# Autodesk Inventor assembly: estação_bga
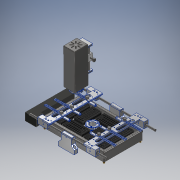
[picture p0: Inventor's stored thumbnail of the model, 180x180]
Saved by Autodesk Inventor 2018 (Build 220112000, 112)
## iProperties
Created: 2018-05-03
Part Number: estação_bga
Material: Genérico
Document SubType Name: Assembly
Designer: Georgines
Author: Georgines
## Documents named in this file (20)
- C:\Users\Usuario\Google Drive\estação bga\pecas_3d\estação_bga.iam
- C:\Users\Usuario\Google Drive\estação bga\pecas_3d\resistencia_original_2.ipt
- C:\Users\Usuario\Google Drive\estação bga\pecas_3d\resistencia_600w.ipt
- C:\Users\Usuario\Google Drive\estação bga\pecas_3d\base_interna_resistencias.ipt
- C:\Users\Usuario\Google Drive\estação bga\pecas_3d\base_externa_resistencias.ipt
- C:\Users\Usuario\Google Drive\estação bga\pecas_3d\tampa_superior_resistencias.ipt
- C:\Users\Usuario\Google Drive\estação bga\pecas_3d\espassador_mesa_resistencias.ipt
- C:\Users\Usuario\Google Drive\estação bga\pecas_3d\ventilador_tangencial_referencia.ipt
- C:\Users\Usuario\Google Drive\estação bga\pecas_3d\chapa_referencia_tampa_gabinete.ipt
- C:\Users\Usuario\Google Drive\estação bga\pecas_3d\suporte_guia_central.ipt
- C:\Users\Usuario\Google Drive\estação bga\pecas_3d\guia_linear_12mm.ipt
- C:\Users\Usuario\Google Drive\estação bga\pecas_3d\rolamento_linear_lm12uu.iam.ipt
- C:\Users\Usuario\Google Drive\estação bga\pecas_3d\carro_do_rolamento_direito.ipt
- C:\Users\Usuario\Google Drive\estação bga\pecas_3d\suporte_pincas.ipt
- C:\Users\Usuario\Google Drive\estação bga\pecas_3d\pinças.ipt
- pinça.ipt
- C:\Users\Usuario\Google Drive\estação bga\pecas_3d\bocal_de_aquecimento.ipt
- C:\Users\Usuario\Google Drive\estação bga\pecas_3d\cabeça_superior.iam
- C:\Users\Usuario\Google Drive\estação bga\pecas_3d\maniplo.ipt
- rolamento_linear_lm12uu.iam
## Components (45 placed, 17 different names)
1. resistencia_original_2:2 — Coincidência:2, Alinhamento:5, Coincidência:4, Alinhamento:7, Alinhamento:8, Alinhamento:11, Coincidência:7
2. resistencia_original_2:3 — Coincidência:1, Alinhamento:1, Alinhamento:2, Coincidência:3, Alinhamento:6, Coincidência:5, Alinhamento:9, Alinhamento:10, Coincidência:6, Alinhamento:14, Alinhamento:15
3. resistencia_original_2:1 — Coincidência:1, Alinhamento:1, Alinhamento:2, Coincidência:2, Alinhamento:5, Alinhamento:8, Alinhamento:9, Alinhamento:13, Alinhamento:16
4. resistencia_original_2:4 — Coincidência:3, Alinhamento:6, Coincidência:4, Alinhamento:7, Coincidência:5, Alinhamento:10, Alinhamento:11
5. resistencia_600w:1 — Coincidência:6, Alinhamento:14, Alinhamento:15, Alinhamento:17
6. resistencia_600w:2 — Coincidência:7, Alinhamento:13, Alinhamento:16
7. base_interna_resistencias:1 — Alinhamento:17, Alinhamento:18, Inserir:15
8. base_externa_resistencias:1 — Alinhamento:18, Alinhamento:19, Alinhamento:20, Inserir:1, Inserir:2, Inserir:3, Inserir:4, Inserir:5, Alinhamento:21, Coincidência:11, Coincidência:12
9. tampa_superior_resistencias:1 — Alinhamento:19
10. espassador_mesa_resistencias — Alinhamento:20
11. espassador_mesa_resistencias:1 — Inserir:4
12. espassador_mesa_resistencias:2 — Inserir:1
13. espassador_mesa_resistencias:3 — Inserir:2
14. espassador_mesa_resistencias:4 — Inserir:3
15. espassador_mesa_resistencias:5 — Inserir:5
16. ventilador_tangencial_referencia:1
17. chapa_referencia_tampa_gabinete:1 — Alinhamento:22
18. suporte_guia_central:1 — Transicional:1, Coincidência:11, Alinhamento:23, Alinhamento:24
19. suporte_guia_central:2 — Coincidência:12, Alinhamento:23, Alinhamento:24, Transicional:9
20. guia_linear_12mm:1 — Transicional:1, Transicional:5, Transicional:6, Alinhamento:25
21. guia_linear_12mm:2 — Transicional:7, Transicional:8, Transicional:9, Alinhamento:25
22. rolamento_linear_lm12uu.iam:1 — Transicional:7, Inserir:7
23. rolamento_linear_lm12uu.iam:2 — Transicional:8, Inserir:9
24. rolamento_linear_lm12uu.iam:3 — Transicional:5, Inserir:8
25. rolamento_linear_lm12uu.iam:4 — Inserir:6, Transicional:6
26. carro_do_rolamento_direito:1 — Inserir:6, Alinhamento:26, Alinhamento:27, Alinhamento:31, Coincidência:13, Alinhamento:33, Coincidência:14
27. carro_do_rolamento_direito:2 — Inserir:7, Alinhamento:26, Alinhamento:27, Alinhamento:31
28. carro_do_rolamento_direito:3 — Inserir:8, Alinhamento:28, Alinhamento:29, Alinhamento:30, Alinhamento:32
29. carro_do_rolamento_direito:4 — Inserir:9, Alinhamento:28, Alinhamento:29, Alinhamento:30
30. suporte_pincas:1 — Alinhamento:32, Coincidência:15, Coincidência:16, Coincidência:17, Coincidência:18, Inserir:10, Inserir:11, Inserir:19, Inserir:20, Inserir:21
31. suporte_pincas:2 — Coincidência:13, Alinhamento:33, Coincidência:14, Coincidência:19, Coincidência:20, Coincidência:21, Inserir:12, Inserir:13, Inserir:14, Inserir:16, Inserir:17, Inserir:18
32. pinça:1 — Coincidência:15, Inserir:10
33. pinça:2 — Coincidência:16, Inserir:11
34. pinça:3 — Coincidência:17, Coincidência:18
35. pinça:4 — Coincidência:19, Inserir:14
36. pinça:5 — Coincidência:20, Inserir:13
37. pinça:6 — Coincidência:21, Inserir:12
38. bocal_de_aquecimento:1 — Inserir:15
39. cabeça_superior:1 [sub-assembly]
40. maniplo:1 — Inserir:16
41. maniplo:2 — Inserir:18
42. maniplo:3 — Inserir:17
43. maniplo:4 — Inserir:21
44. maniplo:5 — Inserir:20
45. maniplo:6 — Inserir:19
## Relationships (75: Flush 30, Insert 21, Mate 18, Transitional 6)
- Coincidência:1 [Mate] (14 mm): resistencia_original_2:3 ↔ resistencia_original_2:1
- Alinhamento:1 [Flush]: resistencia_original_2:3 ↔ resistencia_original_2:1
- Alinhamento:2 [Flush]: resistencia_original_2:3 ↔ resistencia_original_2:1
- Coincidência:2 [Mate] (14 mm): resistencia_original_2:2 ↔ resistencia_original_2:1
- Alinhamento:5 [Flush]: resistencia_original_2:2 ↔ resistencia_original_2:1
- Coincidência:3 [Mate] (14 mm): resistencia_original_2:3 ↔ resistencia_original_2:4
- Alinhamento:6 [Flush]: resistencia_original_2:3 ↔ resistencia_original_2:4
- Coincidência:4 [Mate] (14 mm): resistencia_original_2:2 ↔ resistencia_original_2:4
- Alinhamento:7 [Flush]: resistencia_original_2:2 ↔ resistencia_original_2:4
- Coincidência:5 [Mate] (14 mm): resistencia_original_2:3 ↔ resistencia_original_2:4
- Alinhamento:8 [Flush]: resistencia_original_2:2 ↔ resistencia_original_2:1
- Alinhamento:9 [Flush]: resistencia_original_2:3 ↔ resistencia_original_2:1
- Alinhamento:10 [Flush]: resistencia_original_2:3 ↔ resistencia_original_2:4
- Alinhamento:11 [Flush]: resistencia_original_2:2 ↔ resistencia_original_2:4
- Coincidência:6 [Mate] (10 mm): resistencia_original_2:3 ↔ resistencia_600w:1
- Coincidência:7 [Mate] (10 mm): resistencia_original_2:2 ↔ resistencia_600w:2
- Alinhamento:13 [Flush]: resistencia_original_2:1 ↔ resistencia_600w:2
- Alinhamento:14 [Flush]: resistencia_original_2:3 ↔ resistencia_600w:1
- Alinhamento:15 [Flush]: resistencia_original_2:3 ↔ resistencia_600w:1
- Alinhamento:16 [Flush]: resistencia_original_2:1 ↔ resistencia_600w:2
- Alinhamento:17 [Flush]: resistencia_600w:1 ↔ base_interna_resistencias:1
- Alinhamento:18 [Flush]: base_interna_resistencias:1 ↔ base_externa_resistencias:1
- Alinhamento:19 [Flush]: base_externa_resistencias:1 ↔ tampa_superior_resistencias:1
- Alinhamento:20 [Flush]: base_externa_resistencias:1 ↔ espassador_mesa_resistencias
- Inserir:1: base_externa_resistencias:1 ↔ espassador_mesa_resistencias:2
- Inserir:2: base_externa_resistencias:1 ↔ espassador_mesa_resistencias:3
- Inserir:3: base_externa_resistencias:1 ↔ espassador_mesa_resistencias:4
- Inserir:4: base_externa_resistencias:1 ↔ espassador_mesa_resistencias:1
- Inserir:5: base_externa_resistencias:1 ↔ espassador_mesa_resistencias:5
- Alinhamento:21 [Flush] (8 mm): base_externa_resistencias:1
- Alinhamento:22 [Flush]: chapa_referencia_tampa_gabinete:1
- Transicional:1: suporte_guia_central:1 ↔ guia_linear_12mm:1
- Coincidência:11 [Mate] (20 mm): base_externa_resistencias:1 ↔ suporte_guia_central:1
- Coincidência:12 [Mate] (20 mm): base_externa_resistencias:1 ↔ suporte_guia_central:2
- Alinhamento:23 [Flush]: suporte_guia_central:1 ↔ suporte_guia_central:2
- Alinhamento:24 [Flush]: suporte_guia_central:1 ↔ suporte_guia_central:2
- Transicional:5: guia_linear_12mm:1 ↔ rolamento_linear_lm12uu.iam:3
- Inserir:6: rolamento_linear_lm12uu.iam:4 ↔ carro_do_rolamento_direito:1
- Transicional:6: guia_linear_12mm:1 ↔ rolamento_linear_lm12uu.iam:4
- Transicional:7: guia_linear_12mm:2 ↔ rolamento_linear_lm12uu.iam:1
- Inserir:7: rolamento_linear_lm12uu.iam:1 ↔ carro_do_rolamento_direito:2
- Transicional:8: guia_linear_12mm:2 ↔ rolamento_linear_lm12uu.iam:2
- Transicional:9: suporte_guia_central:2 ↔ guia_linear_12mm:2
- Alinhamento:25 [Flush]: guia_linear_12mm:1 ↔ guia_linear_12mm:2
- Alinhamento:26 [Flush]: carro_do_rolamento_direito:1 ↔ carro_do_rolamento_direito:2
- Alinhamento:27 [Flush]: carro_do_rolamento_direito:1 ↔ carro_do_rolamento_direito:2
- Inserir:8: rolamento_linear_lm12uu.iam:3 ↔ carro_do_rolamento_direito:3
- Inserir:9: rolamento_linear_lm12uu.iam:2 ↔ carro_do_rolamento_direito:4
- Alinhamento:28 [Flush]: carro_do_rolamento_direito:3 ↔ carro_do_rolamento_direito:4
- Alinhamento:29 [Flush]: carro_do_rolamento_direito:3 ↔ carro_do_rolamento_direito:4
- Alinhamento:30 [Flush]: carro_do_rolamento_direito:3 ↔ carro_do_rolamento_direito:4
- Alinhamento:31 [Flush]: carro_do_rolamento_direito:1 ↔ carro_do_rolamento_direito:2
- Alinhamento:32 [Flush]: carro_do_rolamento_direito:3 ↔ suporte_pincas:1
- Coincidência:13 [Mate]: carro_do_rolamento_direito:1 ↔ suporte_pincas:2
- Alinhamento:33 [Flush]: carro_do_rolamento_direito:1 ↔ suporte_pincas:2
- Coincidência:14 [Mate]: carro_do_rolamento_direito:1 ↔ suporte_pincas:2
- Coincidência:15 [Mate]: suporte_pincas:1 ↔ pinça:1
- Coincidência:16 [Mate]: suporte_pincas:1 ↔ pinça:2
- Coincidência:17 [Mate]: suporte_pincas:1 ↔ pinça:3
- Coincidência:18 [Mate]: suporte_pincas:1 ↔ pinça:3
- Inserir:10: suporte_pincas:1 ↔ pinça:1
- Inserir:11: suporte_pincas:1 ↔ pinça:2
- Coincidência:19 [Mate]: suporte_pincas:2 ↔ pinça:4
- Coincidência:20 [Mate]: suporte_pincas:2 ↔ pinça:5
- Coincidência:21 [Mate]: suporte_pincas:2 ↔ pinça:6
- Inserir:12: suporte_pincas:2 ↔ pinça:6
- Inserir:13: suporte_pincas:2 ↔ pinça:5
- Inserir:14: suporte_pincas:2 ↔ pinça:4
- Inserir:15 (-35 mm): base_interna_resistencias:1 ↔ bocal_de_aquecimento:1
- Inserir:16 (-10 mm): suporte_pincas:2 ↔ maniplo:1
- Inserir:17 (-10 mm): suporte_pincas:2 ↔ maniplo:3
- Inserir:18 (-10 mm): suporte_pincas:2 ↔ maniplo:2
- Inserir:19 (-10 mm): suporte_pincas:1 ↔ maniplo:6
- Inserir:20 (-10 mm): suporte_pincas:1 ↔ maniplo:5
- Inserir:21 (-10 mm): suporte_pincas:1 ↔ maniplo:4
